# Autodesk Inventor assembly: Cuvette-Sampleholder-with-base
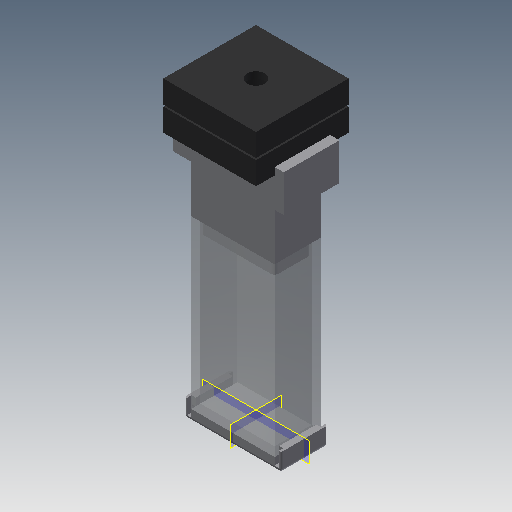
[picture p0: Inventor's stored thumbnail of the model, 512x512]
Saved by Autodesk Inventor 2019 (Build 230136000, 136)
## iProperties
Created: 2020-05-07
Part Number: Cuvette-Sampleholder-with-base
Document SubType Name: Assembly
Designer: voigt
Author: voigt
## Documents named in this file (3)
- C:\Users\nvladi\Documents\Inventor\mesoSPIM_design_benchtop_V2\mesoSPIM\sample_handling\Cuvette-Sampleholder\Cuvette-Sampleholder-with-base.iam
- C:\Users\nvladi\Documents\Inventor\mesoSPIM_design_benchtop_V2\mesoSPIM\sample_handling\Cuvette-Sampleholder\Cuvette-Sampleholder.iam
- C:\Users\nvladi\Documents\Inventor\mesoSPIM_design_benchtop_V2\library\Thorlabs\kinematic_bases\KB25_M-Step.ipt
## Components (2 placed, 2 different names)
1. Cuvette-Sampleholder:1 [sub-assembly] — Mate:1, Mate:2, Angle:1
2. KB25_M-Step:1 — Mate:1, Mate:2, Angle:1
## Relationships (3: Mate 2, Angle 1)
- Mate:1: Cuvette-Sampleholder:1 ↔ KB25_M-Step:1
- Mate:2: Cuvette-Sampleholder:1 ↔ KB25_M-Step:1
- Angle:1 (0 deg): Cuvette-Sampleholder:1 ↔ KB25_M-Step:1
